# Autodesk Inventor assembly: 몸통
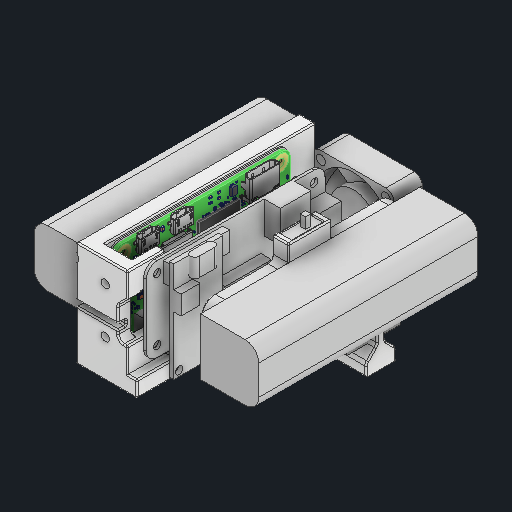
[picture p0: Inventor's stored thumbnail of the model, 512x512]
Saved by Autodesk Inventor 2027.1 (Build 311270010, 270A)
## iProperties
Created: 2026-08-06
Part Number: 몸통
Document SubType Name: Assembly
Designer: moieboy9999
Mass: 235 g
Surface Area: 621.776 cm^2
Volume: 134.898 cm^3
Density: 1.74205 g/cm^3
Author: moieboy9999
## Documents named in this file (9)
- D:\micro_dog_cad\몸\시스템\시스템조립.iam
- D:\micro_dog_cad\부품\배터리+홀더.ipt
- D:\micro_dog_cad\부품\라파+hat.ipt
- D:\micro_dog_cad\부품\스위치.ipt
- D:\micro_dog_cad\부품\BMS.ipt
- D:\micro_dog_cad\부품\충전모듈.ipt
- D:\micro_dog_cad\몸\시스템\마운트.ipt
- D:\micro_dog_cad\부품\팬.ipt
- D:\micro_dog_cad\몸\시스템\Raspberry Pi Zero 2 W.ipt
## Components (9 placed, 8 different names)
1. 라파+hat:1 — 메이트:3, 메이트:17, 메이트:18
2. 스위치:1 — 메이트:12, 메이트:13, 메이트:14
3. 마운트:1 — 메이트:1, 메이트:2, 메이트:3, 메이트:5, 메이트:6, 메이트:7, 메이트:8, 메이트:9, 메이트:10, 메이트:11, 메이트:12, 메이트:13, 메이트:14, 메이트:15, 메이트:16, 메이트:18, 메이트:19, 메이트:20, 메이트:21
4. 배터리+홀더:1 — 메이트:5, 메이트:6
5. 배터리+홀더:2 — 메이트:1, 메이트:2
6. BMS:1 — 메이트:9, 메이트:10, 메이트:11
7. 충전모듈:1 — 메이트:7, 메이트:8
8. 팬:1 — 메이트:15, 메이트:16
9. Raspberry Pi Zero 2 W:1 — 메이트:17, 메이트:19, 메이트:20, 메이트:21
## Relationships (20: Mate 20)
- 메이트:1 [Mate]: 마운트:1 ↔ 배터리+홀더:2
- 메이트:2 [Mate]: 마운트:1 ↔ 배터리+홀더:2
- 메이트:3 [Mate]: 라파+hat:1 ↔ 마운트:1
- 메이트:5 [Mate]: 마운트:1 ↔ 배터리+홀더:1
- 메이트:6 [Mate]: 마운트:1 ↔ 배터리+홀더:1
- 메이트:7 [Mate]: 마운트:1 ↔ 충전모듈:1
- 메이트:8 [Mate]: 마운트:1 ↔ 충전모듈:1
- 메이트:9 [Mate]: 마운트:1 ↔ BMS:1
- 메이트:10 [Mate]: 마운트:1 ↔ BMS:1
- 메이트:11 [Mate]: 마운트:1 ↔ BMS:1
- 메이트:12 [Mate]: 스위치:1 ↔ 마운트:1
- 메이트:13 [Mate]: 스위치:1 ↔ 마운트:1
- 메이트:14 [Mate]: 스위치:1 ↔ 마운트:1
- 메이트:15 [Mate]: 마운트:1 ↔ 팬:1
- 메이트:16 [Mate]: 마운트:1 ↔ 팬:1
- 메이트:17 [Mate]: 라파+hat:1 ↔ Raspberry Pi Zero 2 W:1
- 메이트:18 [Mate]: 라파+hat:1 ↔ 마운트:1
- 메이트:19 [Mate]: 마운트:1 ↔ Raspberry Pi Zero 2 W:1
- 메이트:20 [Mate]: 마운트:1 ↔ Raspberry Pi Zero 2 W:1
- 메이트:21 [Mate]: 마운트:1 ↔ Raspberry Pi Zero 2 W:1
